# Autodesk Inventor assembly: plyta_dmd
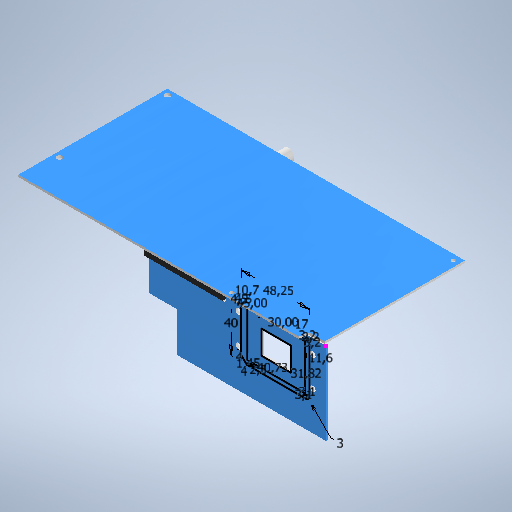
[picture p0: Inventor's stored thumbnail of the model, 512x512]
Saved by Autodesk Inventor 2025.1 (Build 291241000, 241)
## iProperties
Created: 2024-10-24
Part Number: plyta_dmd
Document SubType Name: Assembly
Designer: PC
Author: PC
## Documents named in this file (4)
- C:\Users\PC\Desktop\fotolito_czesci\nowe\plyta_dmd.iam
- C:\Users\PC\Desktop\fotolito_czesci\nowe\daughterboard.ipt
- C:\Users\PC\Desktop\fotolito_czesci\nowe\motherboard.ipt
- C:\Users\PC\Desktop\fotolito_czesci\nowe\podstawka.iam
## Components (3 placed, 3 different names)
1. daughterboard:1 — Zestawiające:1, Równoległe:1, Zestawiające:2
2. motherboard:1 — Zestawiające:1, Równoległe:1, Zestawiające:2
3. podstawka:1 [sub-assembly]
## Relationships (3: Mate 2, Flush 1)
- Zestawiające:1 [Mate] (1.6 mm): daughterboard:1 ↔ motherboard:1
- Równoległe:1 [Flush] (7 mm): daughterboard:1 ↔ motherboard:1
- Zestawiające:2 [Mate]: daughterboard:1 ↔ motherboard:1
